# Autodesk Inventor assembly: A1-19027-400-00 Spool SP-237-2-P-126-1-C
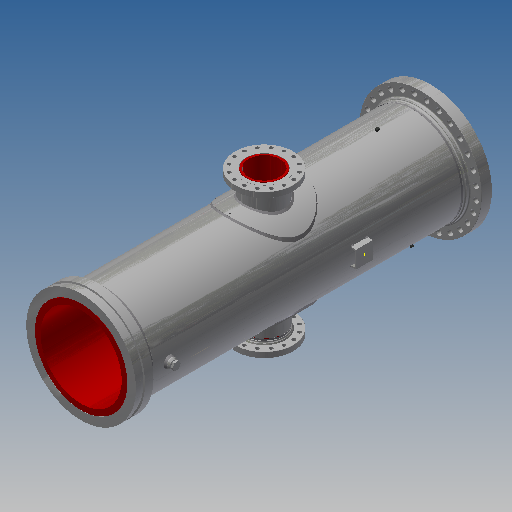
[picture p0: Inventor's stored thumbnail of the model, 512x512]
Saved by Autodesk Inventor 2017.3 (Build 213257000, 257)
## iProperties
Created: 2019-08-16
Part Number: A1-19027-400-00 Spool SP-237-2-P-126-1-C
Document SubType Name: Weldment
Designer: GVD
Weld Material: Steel, Mild, Welded
Mass: 3.29945e+06 g
Surface Area: 380944 cm^2
Volume: 436456 cm^3
Density: 7.55965 g/cm^3
Author: GVD
## Documents named in this file (14)
- N:\A1 - Projects\A1-19\A1-19027--Syncrude Aurora HT2 spools - SP-237\A1-19027-400-00 Spool SP-237-2-P-126-1-C.iam
- N:\A1 - Projects\A1-19\A1-19027--Syncrude Aurora HT2 spools - SP-237\A1-19027-400-02 14in pipe.ipt
- N:\A1 - Projects\A1-19\A1-19027--Syncrude Aurora HT2 spools - SP-237\A1-19027-400-03 Repad.ipt
- N:\A1 - Projects\A1-19\A1-19027--Syncrude Aurora HT2 spools - SP-237\A1-19027-400-05 30in CL300 RF flange.ipt
- N:\A1 - Projects\A1-19\A1-19027--Syncrude Aurora HT2 spools - SP-237\A1-19027-400-07 HCWI liner - trunk.ipt
- N:\A1 - Projects\A1-19\A1-19027--Syncrude Aurora HT2 spools - SP-237\A1-19027-400-09 HCWI liner - drain.ipt
- N:\Inventor\Content Center Files\R2017\en-US\ASME B16.11(23)\ASME B16.11 Hex Head Plug 2.ipt
- N:\Penticton Foundry\Tag mount - 6in.ipt
- N:\A1 - Projects\A1-19\A1-19027--Syncrude Aurora HT2 spools - SP-237\A1-19027-400-01 34in pipe.ipt
- N:\A1 - Projects\A1-19\A1-19027--Syncrude Aurora HT2 spools - SP-237\A1-19027-400-10 2in x 34in threadolet.ipt
- N:\A1 - Projects\A1-19\A1-19027--Syncrude Aurora HT2 spools - SP-237\A1-19027-400-08 HCWI liner - pup.ipt
- N:\A1 - Projects\A1-19\A1-19027--Syncrude Aurora HT2 spools - SP-237\A1-19027-200-02 36in Type B victaulic ring.ipt
- N:\Inventor\Content Center Files\R2017\en-US\ASME B16.11(23)\ASME B16.11 Hex Head Plug 3_4.ipt
- N:\A1 - Projects\A1-19\A1-19027--Syncrude Aurora HT2 spools - SP-237\A1-19027-400-06 12in CL300 RFWN flange.ipt
## Components (20 placed, 13 different names)
1. A1-19027-400-01 34in pipe:1 — Angle:2, Insert:3, Mate:1, Mate:2, Angle:4, Angle:5, Mate:3, Mate:4, Angle:6, Mate:8, Angle:8, Angle:9, Mate:13, Mate:14, Angle:18, Mate:15, Angle:20, Tangent:1, Angle:21, Flush:1, Tangent:2, Insert:13
2. A1-19027-200-02 36in Type B victaulic ring:1 — Insert:3, Insert:5
3. A1-19027-400-05 30in CL300 RF flange:1 — Angle:2, Mate:7, Flush:2, Insert:13
4. A1-19027-400-07 HCWI liner - trunk:1 — Insert:5, Angle:9, Insert:7, Angle:11, Insert:14, Angle:22
5. A1-19027-400-08 HCWI liner - pup:1 — Insert:14, Angle:22
6. A1-19027-400-10 2in x 34in threadolet:1 — Mate:13, Mate:14, Angle:18, Insert:12, Angle:19
7. ASME B16.11 Hex Head Plug 2:1 — Insert:12, Angle:19
8. A1-19027-400-02 14in pipe:1 — Mate:1, Mate:2, Angle:4, Insert:4
9. A1-19027-400-03 Repad:1 — Mate:3, Mate:4, Angle:6
10. A1-19027-400-06 12in CL300 RFWN flange:1 — Insert:4, Angle:5
11. A1-19027-400-09 HCWI liner - drain:1 — Insert:7, Angle:11
12. A1-19027-400-02 14in pipe:2
13. A1-19027-400-03 Repad:2
14. A1-19027-400-06 12in CL300 RFWN flange:2
15. A1-19027-400-09 HCWI liner - drain:2
16. ASME B16.11 Hex Head Plug 3/4:1 — Mate:15, Angle:20, Tangent:1, Angle:21
17. ASME B16.11 Hex Head Plug 3/4:2
18. ASME B16.11 Hex Head Plug 3/4:3
19. Tag mount - 6in:1 — Flush:1, Flush:2, Tangent:2
20. Tag mount - 6in:2
## Component patterns: (2 elements, first: A1-19027-400-02 14in pipe:1 + A1-19027-400-03 Repad:1 + A1-19027-400-06 12in CL300 RFWN flange:1 + A1-19027-400-09 HCWI liner - drain:1), (3 elements, first: ASME B16.11 Hex Head Plug 3/4:1), (2 elements, first: Tag mount - 6in:1)
## Relationships (33: Angle 13, Mate 9, Insert 7, Tangent 2, Flush 2)
- Angle:2 (0 deg): A1-19027-400-01 34in pipe:1 ↔ A1-19027-400-05 30in CL300 RF flange:1
- Insert:3 (2.3813 mm): A1-19027-400-01 34in pipe:1 ↔ A1-19027-200-02 36in Type B victaulic ring:1
- [Angle] (0 deg): A1-19027-400-01 34in pipe:1 ↔ A1-19027-200-02 36in Type B victaulic ring:1
- Mate:1: A1-19027-400-01 34in pipe:1 ↔ A1-19027-400-02 14in pipe:1
- Mate:2: A1-19027-400-01 34in pipe:1 ↔ A1-19027-400-02 14in pipe:1
- Angle:4 (0 deg): A1-19027-400-01 34in pipe:1 ↔ A1-19027-400-02 14in pipe:1
- Insert:4 (2.3813 mm): A1-19027-400-02 14in pipe:1 ↔ A1-19027-400-06 12in CL300 RFWN flange:1
- Angle:5 (0 deg): A1-19027-400-01 34in pipe:1 ↔ A1-19027-400-06 12in CL300 RFWN flange:1
- Mate:3: A1-19027-400-01 34in pipe:1 ↔ A1-19027-400-03 Repad:1
- Mate:4: A1-19027-400-01 34in pipe:1 ↔ A1-19027-400-03 Repad:1
- Angle:6 (0 deg): A1-19027-400-01 34in pipe:1 ↔ A1-19027-400-03 Repad:1
- Mate:7: A1-19027-400-05 30in CL300 RF flange:1
- Mate:8: A1-19027-400-01 34in pipe:1
- Angle:8 (0 deg): A1-19027-400-01 34in pipe:1
- Insert:5: A1-19027-200-02 36in Type B victaulic ring:1 ↔ A1-19027-400-07 HCWI liner - trunk:1
- Angle:9 (0 deg): A1-19027-400-01 34in pipe:1 ↔ A1-19027-400-07 HCWI liner - trunk:1
- Insert:7: A1-19027-400-07 HCWI liner - trunk:1 ↔ A1-19027-400-09 HCWI liner - drain:1
- Angle:11 (0 deg): A1-19027-400-07 HCWI liner - trunk:1 ↔ A1-19027-400-09 HCWI liner - drain:1
- Mate:13: A1-19027-400-01 34in pipe:1 ↔ A1-19027-400-10 2in x 34in threadolet:1
- Mate:14: A1-19027-400-01 34in pipe:1 ↔ A1-19027-400-10 2in x 34in threadolet:1
- Angle:18 (0 deg): A1-19027-400-01 34in pipe:1 ↔ A1-19027-400-10 2in x 34in threadolet:1
- Insert:12 (-15.494 mm): A1-19027-400-10 2in x 34in threadolet:1 ↔ ASME B16.11 Hex Head Plug 2:1
- Angle:19 (0 deg): A1-19027-400-10 2in x 34in threadolet:1 ↔ ASME B16.11 Hex Head Plug 2:1
- Mate:15: A1-19027-400-01 34in pipe:1 ↔ ASME B16.11 Hex Head Plug 3/4:1
- Angle:20 (180 deg): A1-19027-400-01 34in pipe:1 ↔ ASME B16.11 Hex Head Plug 3/4:1
- Tangent:1 (-12.2428 mm): A1-19027-400-01 34in pipe:1 ↔ ASME B16.11 Hex Head Plug 3/4:1
- Angle:21 (0 deg): A1-19027-400-01 34in pipe:1 ↔ ASME B16.11 Hex Head Plug 3/4:1
- Flush:1: A1-19027-400-01 34in pipe:1 ↔ Tag mount - 6in:1
- Flush:2 (990.6 mm): A1-19027-400-05 30in CL300 RF flange:1 ↔ Tag mount - 6in:1
- Tangent:2: A1-19027-400-01 34in pipe:1 ↔ Tag mount - 6in:1
- Insert:13 (2.3813 mm): A1-19027-400-01 34in pipe:1 ↔ A1-19027-400-05 30in CL300 RF flange:1
- Insert:14: A1-19027-400-07 HCWI liner - trunk:1 ↔ A1-19027-400-08 HCWI liner - pup:1
- Angle:22 (0 deg): A1-19027-400-07 HCWI liner - trunk:1 ↔ A1-19027-400-08 HCWI liner - pup:1
